# Autodesk Inventor assembly: CNC1
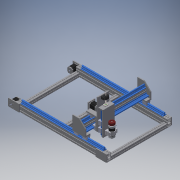
[picture p0: Inventor's stored thumbnail of the model, 180x180]
Saved by Autodesk Inventor 2018 (Build 220112000, 112)
## iProperties
Created: 2018-10-09
Part Number: CNC1
Material: Genérico
Document SubType Name: Assembly
Designer: Georgines
Author: Georgines
## Documents named in this file (30)
- C:\Users\Usuario\Documents\OpenCNC\MONTAGEM\CNC1.iam
- C:\Users\Usuario\Documents\OpenCNC\COMPONENTES_MECANICOS\BLOCOS_GUIAS_LINEARES\SBR16UU.ipt
- C:\Users\Usuario\Documents\OpenCNC\MONTAGEM\CNC1\APOIO_PERFIL_STRUTURAL.ipt
- C:\Users\Usuario\Documents\OpenCNC\MONTAGEM\CNC1\LATERAL_BLOCOS_BASE.ipt
- C:\Users\Usuario\Documents\OpenCNC\MONTAGEM\BLOCO_SUPORTE_EIXO_Z.ipt
- C:\Users\Usuario\Documents\OpenCNC\BAIXADOS\spindle-bldc-500w-1.snapshot.1\SPINDLE_500WSpindle.iam
- C:\Users\Usuario\Documents\OpenCNC\BAIXADOS\spindle-bracket-1.snapshot.2\SUPORTE_SPINDLESpindle Bracket.ipt
- C:\Users\Usuario\Documents\OpenCNC\MONTAGEM\CNC1\BLOCO_SUPORTE_SPINDLE.ipt
- C:\Users\Usuario\Documents\OpenCNC\BAIXADOS\sfu1204-300-with-nut-1.snapshot.3\CASTANHA_FUSO_SFU1204SFU1204-3.ipt
- C:\Users\Usuario\Documents\OpenCNC\BAIXADOS\sfu1204-300-with-nut-1.snapshot.3\FUSO_SFU1204SFU1204-300.ipt
- C:\Users\Usuario\Documents\OpenCNC\BAIXADOS\bearing-support-unit-1.snapshot.1\BK12BK12.ipt
- C:\Users\Usuario\Documents\OpenCNC\BAIXADOS\bearing-support-unit-1.snapshot.1\BF12.ipt
- C:\Users\Usuario\Documents\OpenCNC\COMPONENTES_MECANICOS\GUIAS_LINEARES\SBR16_200MM.ipt
- C:\Users\Usuario\Documents\OpenCNC\COMPONENTES_MECANICOS\PERFIL_ESTRUTURAL\PERFIL_ESTRUTURAL_40X80_EIXO_X.ipt
- C:\Users\Usuario\Documents\OpenCNC\COMPONENTES_MECANICOS\GUIAS_LINEARES\SBR16_EIXO_X_1.ipt
- C:\Users\Usuario\Documents\OpenCNC\COMPONENTES_MECANICOS\GUIAS_LINEARES\SBR16_EIXO_X_2.ipt
- C:\Users\Usuario\Documents\OpenCNC\MONTAGEM\CHAPA_APOIO_INFERIOR_EIXO_X.ipt
- C:\Users\Usuario\Documents\OpenCNC\MONTAGEM\CHAPA_APOIO_SUPERIOR_EIXO_X.ipt
- C:\Users\Usuario\Documents\OpenCNC\BAIXADOS\stepper motor NEMA 23 57x76.ipt
- C:\Users\Usuario\Documents\OpenCNC\MONTAGEM\CHAPA_APOIO_CASTANHA_EIXO_Z.ipt
- C:\Users\Usuario\Documents\OpenCNC\COMPONENTES_MECANICOS\GUIAS_LINEARES\SBR16_EIXO_Y_1.ipt
- C:\Users\Usuario\Documents\OpenCNC\COMPONENTES_MECANICOS\GUIAS_LINEARES\SBR16_EIXO_Y_2.ipt
- C:\Users\Usuario\Documents\OpenCNC\COMPONENTES_MECANICOS\PERFIL_ESTRUTURAL\PERFIL_ESTRUTURAL_40X80_EIXO_Y.ipt
- C:\Users\Usuario\Documents\OpenCNC\COMPONENTES_MECANICOS\PERFIL_ESTRUTURAL\PERFIL_ESTRUTURAL_40X40_EIXO_Y_PERPENDICULAR.ipt
- C:\Users\Usuario\Documents\OpenCNC\MONTAGEM\SUPORTE_MOTOR_EIXO_Y_1.ipt
- C:\Users\Usuario\Documents\OpenCNC\BAIXADOS\stepper motor NEMA 23 57x76_MIR.ipt
- C:\Users\Usuario\Documents\OpenCNC\MONTAGEM\SUPORTE_MOTOR_EIXO_Y_1_MIR.ipt
- C:\Users\Usuario\Documents\OpenCNC\MONTAGEM\SUPORTE_MOTOR_EIXO_X.ipt
- C:\Users\Usuario\Documents\OpenCNC\MONTAGEM\SUPORTE_GUIA_CORREIA_EIXO_Y.ipt
- C:\Users\Usuario\Documents\OpenCNC\MONTAGEM\SUPORTE_GUIA_CORREIA_EIXO_Y_MIR.ipt
## Components (48 placed, 29 different names)
1. SBR16UU:1 — ALINHAMENTO_BOCOS_BASE, ALINHAMENTO_BOCOS_BASE_4, ALINHAMENTO_BOCOS_BASE_6, Alinhamento:32, Alinhamento:33, Coincidência:22, Coincidência:109
2. SBR16UU:2 — ALINHAMENTO_BOCOS_BASE_2, ALINHAMENTO_BOCOS_BASE_4, Alinhamento:31, Alinhamento:149, Coincidência:110
3. SBR16UU:3 — ALINHAMENTO_BOCOS_BASE_2, Alinhamento:81, Alinhamento:148, Coincidência:111
4. SBR16UU:4 — ALINHAMENTO_BOCOS_BASE, ALINHAMENTO_BOCOS_BASE_6, Coincidência:49, Alinhamento:82, Coincidência:108
5. APOIO_PERFIL_STRUTURAL:1 — Alinhamento:31, Alinhamento:32, Alinhamento:33, Coincidência:22, Coincidência:51, Alinhamento:85, Coincidência:86, Alinhamento:149, Alinhamento:177
6. LATERAL_BLOCOS_BASE:1 — Alinhamento:83, Coincidência:51, Alinhamento:85, Coincidência:89, Alinhamento:177
7. BLOCO_SUPORTE_EIXO_Z:1 — Coincidência:66, Coincidência:77, Alinhamento:118, Alinhamento:122, Alinhamento:123, Alinhamento:124, Coincidência:95, Alinhamento:136, Alinhamento:137, Alinhamento:144, Coincidência:98
8. APOIO_PERFIL_STRUTURAL:2 — Coincidência:49, Alinhamento:81, Alinhamento:82, Coincidência:52, Alinhamento:87, Alinhamento:145, Alinhamento:148
9. LATERAL_BLOCOS_BASE:2 — Alinhamento:83, Coincidência:52, Alinhamento:87, Coincidência:88
10. SPINDLE_500WSpindle:1 [sub-assembly] — Coincidência:63, Alinhamento:99
11. SUPORTE_SPINDLESpindle Bracket:1 — Coincidência:62, Alinhamento:97, Alinhamento:98, Coincidência:63, Alinhamento:99
12. BLOCO_SUPORTE_SPINDLE:1 — Coincidência:62, Alinhamento:97, Alinhamento:98, Coincidência:79, Coincidência:81, Alinhamento:119, Alinhamento:120, Alinhamento:121, Alinhamento:151, Alinhamento:152, Alinhamento:153
13. CASTANHA_FUSO_SFU1204SFU1204-3:1 — Coincidência:74, Coincidência:105, Coincidência:106, Coincidência:107
14. BK12BK12:1 — Coincidência:66, Coincidência:72, Alinhamento:101, Alinhamento:103, Alinhamento:124
15. BF12:1 — Coincidência:73, Alinhamento:102, Alinhamento:103, Alinhamento:123
16. FUSO_SFU1204SFU1204-300:2 — Coincidência:72, Alinhamento:101, Coincidência:73, Alinhamento:102, Coincidência:74
17. SBR16UU:9 — Alinhamento:104, Alinhamento:106, Alinhamento:109, Coincidência:75, Coincidência:76, Coincidência:77, Coincidência:78, Alinhamento:122
18. SBR16UU:10 — Alinhamento:104, Alinhamento:107, Alinhamento:108, Alinhamento:109, Coincidência:76, Coincidência:80
19. SBR16UU:11 — Alinhamento:105, Alinhamento:106, Alinhamento:110, Coincidência:75
20. SBR16UU:12 — Alinhamento:105, Alinhamento:107, Alinhamento:108, Alinhamento:110, Alinhamento:118
21. SBR16_200MM:1 — Coincidência:78, Coincidência:79, Alinhamento:119, Alinhamento:121
22. SBR16_200MM:2 — Coincidência:80, Coincidência:81, Alinhamento:120
23. PERFIL_ESTRUTURAL_40X80_EIXO_X:1 — Alinhamento:127, Coincidência:86, Coincidência:88, Coincidência:89, Coincidência:90, Alinhamento:134, Alinhamento:145, Coincidência:112, Alinhamento:155
24. SBR16_EIXO_X_1:1 — Alinhamento:127, Coincidência:90, Alinhamento:134, Coincidência:91, Coincidência:92, Alinhamento:156
25. SBR16UU:13 — Coincidência:91, Alinhamento:143, Coincidência:100
26. SBR16UU:14 — Coincidência:92, Alinhamento:142, Coincidência:99
27. SBR16UU:15 — Coincidência:96, Coincidência:126, Alinhamento:173, Alinhamento:175
28. SBR16UU:16 — Coincidência:97, Alinhamento:138, Alinhamento:140, Coincidência:113
29. CHAPA_APOIO_INFERIOR_EIXO_X:1 — Coincidência:95, Alinhamento:136, Alinhamento:137, Coincidência:96, Coincidência:97, Alinhamento:138, Alinhamento:140, Alinhamento:141, Alinhamento:174, Alinhamento:175
30. CHAPA_APOIO_SUPERIOR_EIXO_X:1 — Alinhamento:141, Alinhamento:142, Alinhamento:143, Alinhamento:144, Coincidência:98, Coincidência:99, Coincidência:100, Coincidência:104, Coincidência:129, Alinhamento:176
31. stepper motor NEMA 23 57x76:1 — Coincidência:104, Coincidência:128, Ângulo:3, Coincidência:130
32. CHAPA_APOIO_CASTANHA_EIXO_Z:1 — Alinhamento:151, Alinhamento:152, Alinhamento:153, Coincidência:105, Coincidência:106, Coincidência:107
33. SBR16_EIXO_Y_1:1 — Coincidência:109, Coincidência:110, Alinhamento:154, Alinhamento:157, Coincidência:115, Alinhamento:158, Alinhamento:159
34. SBR16_EIXO_Y_2:1 — Coincidência:108, Coincidência:111, Alinhamento:154, Alinhamento:157, Coincidência:116, Alinhamento:160, Alinhamento:161
35. SBR16_EIXO_X_2:1 — Coincidência:112, Alinhamento:155, Alinhamento:156, Coincidência:113, Coincidência:126, Coincidência:127
36. PERFIL_ESTRUTURAL_40X80_EIXO_Y:1 — Coincidência:115, Alinhamento:158, Alinhamento:159, Alinhamento:164, Alinhamento:165, Alinhamento:166, Coincidência:122, Coincidência:131, Coincidência:133, Alinhamento:180, Coincidência:135, Coincidência:136, Alinhamento:183, Alinhamento:184
37. PERFIL_ESTRUTURAL_40X80_EIXO_Y:2 — Coincidência:116, Alinhamento:160, Alinhamento:161, Coincidência:117, Alinhamento:162, Alinhamento:163, Coincidência:118, Coincidência:119, Coincidência:125, Coincidência:132, Alinhamento:181, Coincidência:137, Alinhamento:185, Alinhamento:186
38. PERFIL_ESTRUTURAL_40X40_EIXO_Y_PERPENDICULAR:1 — Coincidência:117, Alinhamento:162, Alinhamento:163
39. PERFIL_ESTRUTURAL_40X40_EIXO_Y_PERPENDICULAR:2 — Coincidência:118, Alinhamento:164, Alinhamento:165, Alinhamento:167
40. PERFIL_ESTRUTURAL_40X40_EIXO_Y_PERPENDICULAR:3 — Coincidência:119, Alinhamento:166, Alinhamento:167
41. stepper motor NEMA 23 57x76:3 — Coincidência:120, Ângulo:1, Coincidência:121, Coincidência:135
42. SUPORTE_MOTOR_EIXO_Y_1:1 — Coincidência:120, Ângulo:1, Coincidência:121, Coincidência:122, Alinhamento:180, Alinhamento:182
43. stepper motor NEMA 23 57x76_MIR:1 — Coincidência:123, Ângulo:2, Coincidência:124
44. SUPORTE_MOTOR_EIXO_Y_1_MIR:1 — Coincidência:123, Ângulo:2, Coincidência:124, Coincidência:125, Alinhamento:181, Alinhamento:182
45. SBR16UU:17 — Coincidência:127, Alinhamento:173, Alinhamento:174
46. SUPORTE_MOTOR_EIXO_X:1 — Coincidência:128, Ângulo:3, Coincidência:129, Coincidência:130, Alinhamento:176
47. SUPORTE_GUIA_CORREIA_EIXO_Y:1 — Coincidência:136, Alinhamento:183, Alinhamento:184
48. SUPORTE_GUIA_CORREIA_EIXO_Y_MIR:1 — Coincidência:137, Alinhamento:185, Alinhamento:186
## Relationships (138: Flush 74, Mate 61, Angle 3)
- ALINHAMENTO_BOCOS_BASE [Flush]: SBR16UU:1 ↔ SBR16UU:4
- ALINHAMENTO_BOCOS_BASE_2 [Flush]: SBR16UU:2 ↔ SBR16UU:3
- ALINHAMENTO_BOCOS_BASE_4 [Flush]: SBR16UU:1 ↔ SBR16UU:2
- ALINHAMENTO_BOCOS_BASE_6 [Flush]: SBR16UU:1 ↔ SBR16UU:4
- Alinhamento:31 [Flush]: SBR16UU:2 ↔ APOIO_PERFIL_STRUTURAL:1
- Alinhamento:32 [Flush]: SBR16UU:1 ↔ APOIO_PERFIL_STRUTURAL:1
- Alinhamento:33 [Flush]: SBR16UU:1 ↔ APOIO_PERFIL_STRUTURAL:1
- Coincidência:22 [Mate]: SBR16UU:1 ↔ APOIO_PERFIL_STRUTURAL:1
- Coincidência:49 [Mate]: SBR16UU:4 ↔ APOIO_PERFIL_STRUTURAL:2
- Alinhamento:81 [Flush]: SBR16UU:3 ↔ APOIO_PERFIL_STRUTURAL:2
- Alinhamento:82 [Flush]: SBR16UU:4 ↔ APOIO_PERFIL_STRUTURAL:2
- Alinhamento:83 [Flush]: LATERAL_BLOCOS_BASE:1 ↔ LATERAL_BLOCOS_BASE:2
- Coincidência:51 [Mate]: APOIO_PERFIL_STRUTURAL:1 ↔ LATERAL_BLOCOS_BASE:1
- Alinhamento:85 [Flush]: APOIO_PERFIL_STRUTURAL:1 ↔ LATERAL_BLOCOS_BASE:1
- Coincidência:52 [Mate]: APOIO_PERFIL_STRUTURAL:2 ↔ LATERAL_BLOCOS_BASE:2
- Alinhamento:87 [Flush]: APOIO_PERFIL_STRUTURAL:2 ↔ LATERAL_BLOCOS_BASE:2
- Coincidência:62 [Mate]: SUPORTE_SPINDLESpindle Bracket:1 ↔ BLOCO_SUPORTE_SPINDLE:1
- Alinhamento:97 [Flush] (25 mm): SUPORTE_SPINDLESpindle Bracket:1 ↔ BLOCO_SUPORTE_SPINDLE:1
- Alinhamento:98 [Flush] (18 mm): SUPORTE_SPINDLESpindle Bracket:1 ↔ BLOCO_SUPORTE_SPINDLE:1
- Coincidência:63 [Mate]: SPINDLE_500WSpindle:1 ↔ SUPORTE_SPINDLESpindle Bracket:1
- Alinhamento:99 [Flush] (-25 mm): SPINDLE_500WSpindle:1 ↔ SUPORTE_SPINDLESpindle Bracket:1
- Coincidência:66 [Mate]: BLOCO_SUPORTE_EIXO_Z:1 ↔ BK12BK12:1
- Coincidência:72 [Mate]: BK12BK12:1 ↔ FUSO_SFU1204SFU1204-300:2
- Alinhamento:101 [Flush] (18.31 mm): BK12BK12:1 ↔ FUSO_SFU1204SFU1204-300:2
- Coincidência:73 [Mate]: BF12:1 ↔ FUSO_SFU1204SFU1204-300:2
- Alinhamento:102 [Flush] (-1.5 mm): BF12:1 ↔ FUSO_SFU1204SFU1204-300:2
- Alinhamento:103 [Flush]: BK12BK12:1 ↔ BF12:1
- Coincidência:74 [Mate]: CASTANHA_FUSO_SFU1204SFU1204-3:1 ↔ FUSO_SFU1204SFU1204-300:2
- Alinhamento:104 [Flush]: SBR16UU:9 ↔ SBR16UU:10
- Alinhamento:105 [Flush]: SBR16UU:11 ↔ SBR16UU:12
- Alinhamento:106 [Flush]: SBR16UU:9 ↔ SBR16UU:11
- Alinhamento:107 [Flush]: SBR16UU:10 ↔ SBR16UU:12
- Alinhamento:108 [Flush]: SBR16UU:10 ↔ SBR16UU:12
- Alinhamento:109 [Flush]: SBR16UU:9 ↔ SBR16UU:10
- Alinhamento:110 [Flush]: SBR16UU:11 ↔ SBR16UU:12
- Coincidência:75 [Mate] (23 mm): SBR16UU:9 ↔ SBR16UU:11
- Coincidência:76 [Mate] (35 mm): SBR16UU:9 ↔ SBR16UU:10
- Coincidência:77 [Mate]: BLOCO_SUPORTE_EIXO_Z:1 ↔ SBR16UU:9
- Alinhamento:118 [Flush]: BLOCO_SUPORTE_EIXO_Z:1 ↔ SBR16UU:12
- Coincidência:78 [Mate]: SBR16UU:9 ↔ SBR16_200MM:1
- Coincidência:79 [Mate]: BLOCO_SUPORTE_SPINDLE:1 ↔ SBR16_200MM:1
- Coincidência:80 [Mate]: SBR16UU:10 ↔ SBR16_200MM:2
- Coincidência:81 [Mate]: BLOCO_SUPORTE_SPINDLE:1 ↔ SBR16_200MM:2
- Alinhamento:119 [Flush]: BLOCO_SUPORTE_SPINDLE:1 ↔ SBR16_200MM:1
- Alinhamento:120 [Flush]: BLOCO_SUPORTE_SPINDLE:1 ↔ SBR16_200MM:2
- Alinhamento:121 [Flush] (-2.5 mm): BLOCO_SUPORTE_SPINDLE:1 ↔ SBR16_200MM:1
- Alinhamento:122 [Flush]: BLOCO_SUPORTE_EIXO_Z:1 ↔ SBR16UU:9
- Alinhamento:123 [Flush] (46.627 mm): BLOCO_SUPORTE_EIXO_Z:1 ↔ BF12:1
- Alinhamento:124 [Flush] (32.5 mm): BLOCO_SUPORTE_EIXO_Z:1 ↔ BK12BK12:1
- Alinhamento:127 [Flush]: PERFIL_ESTRUTURAL_40X80_EIXO_X:1 ↔ SBR16_EIXO_X_1:1
- Coincidência:86 [Mate]: APOIO_PERFIL_STRUTURAL:1 ↔ PERFIL_ESTRUTURAL_40X80_EIXO_X:1
- Coincidência:88 [Mate]: LATERAL_BLOCOS_BASE:2 ↔ PERFIL_ESTRUTURAL_40X80_EIXO_X:1
- Coincidência:89 [Mate]: LATERAL_BLOCOS_BASE:1 ↔ PERFIL_ESTRUTURAL_40X80_EIXO_X:1
- Coincidência:90 [Mate]: PERFIL_ESTRUTURAL_40X80_EIXO_X:1 ↔ SBR16_EIXO_X_1:1
- Alinhamento:134 [Flush]: PERFIL_ESTRUTURAL_40X80_EIXO_X:1 ↔ SBR16_EIXO_X_1:1
- Coincidência:91 [Mate]: SBR16_EIXO_X_1:1 ↔ SBR16UU:13
- Coincidência:92 [Mate]: SBR16_EIXO_X_1:1 ↔ SBR16UU:14
- Coincidência:95 [Mate]: BLOCO_SUPORTE_EIXO_Z:1 ↔ CHAPA_APOIO_INFERIOR_EIXO_X:1
- Alinhamento:136 [Flush]: BLOCO_SUPORTE_EIXO_Z:1 ↔ CHAPA_APOIO_INFERIOR_EIXO_X:1
- Alinhamento:137 [Flush]: BLOCO_SUPORTE_EIXO_Z:1 ↔ CHAPA_APOIO_INFERIOR_EIXO_X:1
- Coincidência:96 [Mate]: SBR16UU:15 ↔ CHAPA_APOIO_INFERIOR_EIXO_X:1
- Coincidência:97 [Mate]: SBR16UU:16 ↔ CHAPA_APOIO_INFERIOR_EIXO_X:1
- Alinhamento:138 [Flush]: SBR16UU:16 ↔ CHAPA_APOIO_INFERIOR_EIXO_X:1
- Alinhamento:140 [Flush]: SBR16UU:16 ↔ CHAPA_APOIO_INFERIOR_EIXO_X:1
- Alinhamento:141 [Flush]: CHAPA_APOIO_INFERIOR_EIXO_X:1 ↔ CHAPA_APOIO_SUPERIOR_EIXO_X:1
- Alinhamento:142 [Flush]: SBR16UU:14 ↔ CHAPA_APOIO_SUPERIOR_EIXO_X:1
- Alinhamento:143 [Flush]: SBR16UU:13 ↔ CHAPA_APOIO_SUPERIOR_EIXO_X:1
- Alinhamento:144 [Flush]: BLOCO_SUPORTE_EIXO_Z:1 ↔ CHAPA_APOIO_SUPERIOR_EIXO_X:1
- Coincidência:98 [Mate]: BLOCO_SUPORTE_EIXO_Z:1 ↔ CHAPA_APOIO_SUPERIOR_EIXO_X:1
- Alinhamento:145 [Flush] (-55 mm): APOIO_PERFIL_STRUTURAL:2 ↔ PERFIL_ESTRUTURAL_40X80_EIXO_X:1
- Coincidência:99 [Mate]: SBR16UU:14 ↔ CHAPA_APOIO_SUPERIOR_EIXO_X:1
- Coincidência:100 [Mate]: SBR16UU:13 ↔ CHAPA_APOIO_SUPERIOR_EIXO_X:1
- Alinhamento:148 [Flush]: SBR16UU:3 ↔ APOIO_PERFIL_STRUTURAL:2
- Alinhamento:149 [Flush]: SBR16UU:2 ↔ APOIO_PERFIL_STRUTURAL:1
- Coincidência:104 [Mate]: CHAPA_APOIO_SUPERIOR_EIXO_X:1 ↔ stepper motor NEMA 23 57x76:1
- Alinhamento:151 [Flush]: BLOCO_SUPORTE_SPINDLE:1 ↔ CHAPA_APOIO_CASTANHA_EIXO_Z:1
- Alinhamento:152 [Flush]: BLOCO_SUPORTE_SPINDLE:1 ↔ CHAPA_APOIO_CASTANHA_EIXO_Z:1
- Alinhamento:153 [Flush]: BLOCO_SUPORTE_SPINDLE:1 ↔ CHAPA_APOIO_CASTANHA_EIXO_Z:1
- Coincidência:105 [Mate]: CASTANHA_FUSO_SFU1204SFU1204-3:1 ↔ CHAPA_APOIO_CASTANHA_EIXO_Z:1
- Coincidência:106 [Mate]: CASTANHA_FUSO_SFU1204SFU1204-3:1 ↔ CHAPA_APOIO_CASTANHA_EIXO_Z:1
- Coincidência:107 [Mate]: CASTANHA_FUSO_SFU1204SFU1204-3:1 ↔ CHAPA_APOIO_CASTANHA_EIXO_Z:1
- Coincidência:108 [Mate]: SBR16UU:4 ↔ SBR16_EIXO_Y_2:1
- Coincidência:109 [Mate]: SBR16UU:1 ↔ SBR16_EIXO_Y_1:1
- Coincidência:110 [Mate]: SBR16UU:2 ↔ SBR16_EIXO_Y_1:1
- Coincidência:111 [Mate]: SBR16UU:3 ↔ SBR16_EIXO_Y_2:1
- Alinhamento:154 [Flush]: SBR16_EIXO_Y_1:1 ↔ SBR16_EIXO_Y_2:1
- Coincidência:112 [Mate]: PERFIL_ESTRUTURAL_40X80_EIXO_X:1 ↔ SBR16_EIXO_X_2:1
- Alinhamento:155 [Flush]: PERFIL_ESTRUTURAL_40X80_EIXO_X:1 ↔ SBR16_EIXO_X_2:1
- Alinhamento:156 [Flush]: SBR16_EIXO_X_1:1 ↔ SBR16_EIXO_X_2:1
- Coincidência:113 [Mate]: SBR16UU:16 ↔ SBR16_EIXO_X_2:1
- Alinhamento:157 [Flush]: SBR16_EIXO_Y_1:1 ↔ SBR16_EIXO_Y_2:1
- Coincidência:115 [Mate]: SBR16_EIXO_Y_1:1 ↔ PERFIL_ESTRUTURAL_40X80_EIXO_Y:1
- Coincidência:116 [Mate]: SBR16_EIXO_Y_2:1 ↔ PERFIL_ESTRUTURAL_40X80_EIXO_Y:2
- Alinhamento:158 [Flush] (50 mm): SBR16_EIXO_Y_1:1 ↔ PERFIL_ESTRUTURAL_40X80_EIXO_Y:1
- Alinhamento:159 [Flush]: SBR16_EIXO_Y_1:1 ↔ PERFIL_ESTRUTURAL_40X80_EIXO_Y:1
- Alinhamento:160 [Flush] (50 mm): SBR16_EIXO_Y_2:1 ↔ PERFIL_ESTRUTURAL_40X80_EIXO_Y:2
- Alinhamento:161 [Flush]: SBR16_EIXO_Y_2:1 ↔ PERFIL_ESTRUTURAL_40X80_EIXO_Y:2
- Coincidência:117 [Mate]: PERFIL_ESTRUTURAL_40X80_EIXO_Y:2 ↔ PERFIL_ESTRUTURAL_40X40_EIXO_Y_PERPENDICULAR:1
- Alinhamento:162 [Flush]: PERFIL_ESTRUTURAL_40X80_EIXO_Y:2 ↔ PERFIL_ESTRUTURAL_40X40_EIXO_Y_PERPENDICULAR:1
- Alinhamento:163 [Flush]: PERFIL_ESTRUTURAL_40X80_EIXO_Y:2 ↔ PERFIL_ESTRUTURAL_40X40_EIXO_Y_PERPENDICULAR:1
- Coincidência:118 [Mate]: PERFIL_ESTRUTURAL_40X80_EIXO_Y:2 ↔ PERFIL_ESTRUTURAL_40X40_EIXO_Y_PERPENDICULAR:2
- Alinhamento:164 [Flush]: PERFIL_ESTRUTURAL_40X80_EIXO_Y:1 ↔ PERFIL_ESTRUTURAL_40X40_EIXO_Y_PERPENDICULAR:2
- Alinhamento:165 [Flush]: PERFIL_ESTRUTURAL_40X80_EIXO_Y:1 ↔ PERFIL_ESTRUTURAL_40X40_EIXO_Y_PERPENDICULAR:2
- Coincidência:119 [Mate]: PERFIL_ESTRUTURAL_40X80_EIXO_Y:2 ↔ PERFIL_ESTRUTURAL_40X40_EIXO_Y_PERPENDICULAR:3
- Alinhamento:166 [Flush]: PERFIL_ESTRUTURAL_40X80_EIXO_Y:1 ↔ PERFIL_ESTRUTURAL_40X40_EIXO_Y_PERPENDICULAR:3
- Alinhamento:167 [Flush] (-433.419 mm): PERFIL_ESTRUTURAL_40X40_EIXO_Y_PERPENDICULAR:2 ↔ PERFIL_ESTRUTURAL_40X40_EIXO_Y_PERPENDICULAR:3
- Coincidência:120 [Mate]: stepper motor NEMA 23 57x76:3 ↔ SUPORTE_MOTOR_EIXO_Y_1:1
- Ângulo:1 [Angle] (0 deg): stepper motor NEMA 23 57x76:3 ↔ SUPORTE_MOTOR_EIXO_Y_1:1
- Coincidência:121 [Mate]: stepper motor NEMA 23 57x76:3 ↔ SUPORTE_MOTOR_EIXO_Y_1:1
- Coincidência:122 [Mate]: PERFIL_ESTRUTURAL_40X80_EIXO_Y:1 ↔ SUPORTE_MOTOR_EIXO_Y_1:1
- Coincidência:123 [Mate]: stepper motor NEMA 23 57x76_MIR:1 ↔ SUPORTE_MOTOR_EIXO_Y_1_MIR:1
- Ângulo:2 [Angle] (0 deg): stepper motor NEMA 23 57x76_MIR:1 ↔ SUPORTE_MOTOR_EIXO_Y_1_MIR:1
- Coincidência:124 [Mate]: stepper motor NEMA 23 57x76_MIR:1 ↔ SUPORTE_MOTOR_EIXO_Y_1_MIR:1
- Coincidência:125 [Mate]: PERFIL_ESTRUTURAL_40X80_EIXO_Y:2 ↔ SUPORTE_MOTOR_EIXO_Y_1_MIR:1
- Coincidência:126 [Mate]: SBR16UU:15 ↔ SBR16_EIXO_X_2:1
- Coincidência:127 [Mate]: SBR16_EIXO_X_2:1 ↔ SBR16UU:17
- Alinhamento:173 [Flush]: SBR16UU:15 ↔ SBR16UU:17
- Alinhamento:174 [Flush]: CHAPA_APOIO_INFERIOR_EIXO_X:1 ↔ SBR16UU:17
- Alinhamento:175 [Flush]: SBR16UU:15 ↔ CHAPA_APOIO_INFERIOR_EIXO_X:1
- Coincidência:128 [Mate]: stepper motor NEMA 23 57x76:1 ↔ SUPORTE_MOTOR_EIXO_X:1
- Ângulo:3 [Angle] (0 deg): stepper motor NEMA 23 57x76:1 ↔ SUPORTE_MOTOR_EIXO_X:1
- Coincidência:129 [Mate]: CHAPA_APOIO_SUPERIOR_EIXO_X:1 ↔ SUPORTE_MOTOR_EIXO_X:1
- Coincidência:130 [Mate]: stepper motor NEMA 23 57x76:1 ↔ SUPORTE_MOTOR_EIXO_X:1
- Alinhamento:176 [Flush] (-25 mm): CHAPA_APOIO_SUPERIOR_EIXO_X:1 ↔ SUPORTE_MOTOR_EIXO_X:1
- Coincidência:131 [Mate]: PERFIL_ESTRUTURAL_40X80_EIXO_Y:1
- Coincidência:132 [Mate]: PERFIL_ESTRUTURAL_40X80_EIXO_Y:2
- Coincidência:133 [Mate]: PERFIL_ESTRUTURAL_40X80_EIXO_Y:1
- Alinhamento:177 [Flush]: APOIO_PERFIL_STRUTURAL:1 ↔ LATERAL_BLOCOS_BASE:1
- Alinhamento:180 [Flush]: PERFIL_ESTRUTURAL_40X80_EIXO_Y:1 ↔ SUPORTE_MOTOR_EIXO_Y_1:1
- Alinhamento:181 [Flush]: PERFIL_ESTRUTURAL_40X80_EIXO_Y:2 ↔ SUPORTE_MOTOR_EIXO_Y_1_MIR:1
- Alinhamento:182 [Flush]: SUPORTE_MOTOR_EIXO_Y_1:1 ↔ SUPORTE_MOTOR_EIXO_Y_1_MIR:1
- Coincidência:135 [Mate] (10 mm): PERFIL_ESTRUTURAL_40X80_EIXO_Y:1 ↔ stepper motor NEMA 23 57x76:3
- Coincidência:136 [Mate]: PERFIL_ESTRUTURAL_40X80_EIXO_Y:1 ↔ SUPORTE_GUIA_CORREIA_EIXO_Y:1
- Alinhamento:183 [Flush]: PERFIL_ESTRUTURAL_40X80_EIXO_Y:1 ↔ SUPORTE_GUIA_CORREIA_EIXO_Y:1
- Alinhamento:184 [Flush]: PERFIL_ESTRUTURAL_40X80_EIXO_Y:1 ↔ SUPORTE_GUIA_CORREIA_EIXO_Y:1
- Coincidência:137 [Mate]: PERFIL_ESTRUTURAL_40X80_EIXO_Y:2 ↔ SUPORTE_GUIA_CORREIA_EIXO_Y_MIR:1
- Alinhamento:185 [Flush]: PERFIL_ESTRUTURAL_40X80_EIXO_Y:2 ↔ SUPORTE_GUIA_CORREIA_EIXO_Y_MIR:1
- Alinhamento:186 [Flush]: PERFIL_ESTRUTURAL_40X80_EIXO_Y:2 ↔ SUPORTE_GUIA_CORREIA_EIXO_Y_MIR:1
